# Autodesk Inventor assembly: main body assembly
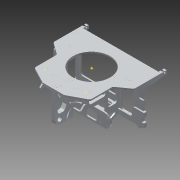
[picture p0: Inventor's stored thumbnail of the model, 180x180]
Saved by Autodesk Inventor 2015 (Build 190159000, 159)
## iProperties
Created: 2015-08-16
Part Number: main body assembly
Document SubType Name: Assembly
Designer: Thomas
Author: Thomas
## Documents named in this file (10)
- C:\Users\Thomas\Google Drive\MSc ROBOTICS\PROJECT\OpenROV\openrov-hardware\CAD_Files_OpenROV_v2_5\main body assembly.iam
- C:\Users\Thomas\Google Drive\MSc ROBOTICS\PROJECT\OpenROV\openrov-hardware\CAD_Files_OpenROV_v2_5\Internal Structure\Bulkhead 25083113.ipt
- C:\Users\Thomas\Google Drive\MSc ROBOTICS\PROJECT\OpenROV\openrov-hardware\CAD_Files_OpenROV_v2_5\Internal Structure\Axial Shroud Support 25090213.ipt
- C:\Users\Thomas\Google Drive\MSc ROBOTICS\PROJECT\OpenROV\openrov-hardware\CAD_Files_OpenROV_v2_5\Internal Structure\Bulkhead Brace 25100613.ipt
- C:\Users\Thomas\Google Drive\MSc ROBOTICS\PROJECT\OpenROV\openrov-hardware\CAD_Files_OpenROV_v2_5\Internal Structure\Vertical Motor Mount 25090213.ipt
- C:\Users\Thomas\Google Drive\MSc ROBOTICS\PROJECT\OpenROV\openrov-hardware\CAD_Files_OpenROV_v2_5\Internal Structure\Horizontal Motor Mount 25090213.ipt
- C:\Users\Thomas\Google Drive\MSc ROBOTICS\PROJECT\OpenROV\openrov-hardware\CAD_Files_OpenROV_v2_5\Internal Structure\Handle 25090213.ipt
- C:\Users\Thomas\Google Drive\MSc ROBOTICS\PROJECT\OpenROV\openrov-hardware\CAD_Files_OpenROV_v2_5\Internal Structure\Lateral Shroud Support 25090213.ipt
- C:\Users\Thomas\Google Drive\MSc ROBOTICS\PROJECT\OpenROV\openrov-hardware\CAD_Files_OpenROV_v2_5\Internal Structure\Top Plate 25090213.ipt
- C:\Users\Thomas\Google Drive\MSc ROBOTICS\PROJECT\OpenROV\openrov-hardware\CAD_Files_OpenROV_v2_5\Internal Structure\Tube Cradle 25090213.ipt
## Components (15 placed, 9 different names)
1. Bulkhead 25083113:1
2. Axial Shroud Support 25090213:1
3. Axial Shroud Support 25090213:2
4. Bulkhead Brace 25100613:1
5. Vertical Motor Mount 25090213:1
6. Horizontal Motor Mount 25090213:1
7. Handle 25090213:1
8. Handle 25090213:2
9. Handle 25090213:3
10. Lateral Shroud Support 25090213:1
11. Top Plate 25090213:1
12. Tube Cradle 25090213:1
13. Tube Cradle 25090213:2
14. Tube Cradle 25090213:3
15. Tube Cradle 25090213:4
## Relationships (42: Mate 31, Flush 11)
- [Mate]: Bulkhead 25083113:1 ↔ Axial Shroud Support 25090213:1
- [Mate]: Bulkhead 25083113:1 ↔ Axial Shroud Support 25090213:1
- [Mate]: Bulkhead 25083113:1 ↔ Axial Shroud Support 25090213:1
- [Mate]: Bulkhead 25083113:1 ↔ Axial Shroud Support 25090213:2
- [Mate]: Bulkhead 25083113:1 ↔ Axial Shroud Support 25090213:2
- [Mate]: Bulkhead 25083113:1 ↔ Axial Shroud Support 25090213:2
- [Mate]: Bulkhead 25083113:1 ↔ Bulkhead Brace 25100613:1
- [Flush]: Bulkhead 25083113:1 ↔ Bulkhead Brace 25100613:1
- [Flush]: Bulkhead 25083113:1 ↔ Bulkhead Brace 25100613:1
- [Mate]: Bulkhead 25083113:1 ↔ Vertical Motor Mount 25090213:1
- [Mate]: Bulkhead 25083113:1 ↔ Vertical Motor Mount 25090213:1
- [Mate]: Bulkhead 25083113:1 ↔ Vertical Motor Mount 25090213:1
- [Mate]: Vertical Motor Mount 25090213:1 ↔ Horizontal Motor Mount 25090213:1
- [Mate]: Vertical Motor Mount 25090213:1 ↔ Horizontal Motor Mount 25090213:1
- [Mate]: Vertical Motor Mount 25090213:1 ↔ Horizontal Motor Mount 25090213:1
- [Mate]: Handle 25090213:1 ↔ Handle 25090213:2
- [Flush]: Handle 25090213:1 ↔ Handle 25090213:2
- [Flush]: Handle 25090213:1 ↔ Handle 25090213:2
- [Mate]: Handle 25090213:2 ↔ Handle 25090213:3
- [Flush]: Handle 25090213:2 ↔ Handle 25090213:3
- [Flush]: Handle 25090213:2 ↔ Handle 25090213:3
- [Mate]: Handle 25090213:2 ↔ Lateral Shroud Support 25090213:1
- [Mate]: Handle 25090213:1 ↔ Lateral Shroud Support 25090213:1
- [Mate]: Handle 25090213:2 ↔ Lateral Shroud Support 25090213:1
- [Mate]: Handle 25090213:2 ↔ Top Plate 25090213:1
- [Flush]: Handle 25090213:2 ↔ Top Plate 25090213:1
- [Mate]: Handle 25090213:3 ↔ Top Plate 25090213:1
- [Mate]: Bulkhead 25083113:1 ↔ Top Plate 25090213:1
- [Mate]: Bulkhead 25083113:1 ↔ Top Plate 25090213:1
- [Mate]: Bulkhead 25083113:1 ↔ Top Plate 25090213:1
- [Mate]: Tube Cradle 25090213:1 ↔ Tube Cradle 25090213:2
- [Flush]: Tube Cradle 25090213:1 ↔ Tube Cradle 25090213:2
- [Flush]: Tube Cradle 25090213:1 ↔ Tube Cradle 25090213:2
- [Mate]: Tube Cradle 25090213:3 ↔ Tube Cradle 25090213:4
- [Flush]: Tube Cradle 25090213:3 ↔ Tube Cradle 25090213:4
- [Flush]: Tube Cradle 25090213:3 ↔ Tube Cradle 25090213:4
- [Mate]: Top Plate 25090213:1 ↔ Tube Cradle 25090213:2
- [Mate]: Bulkhead 25083113:1 ↔ Tube Cradle 25090213:2
- [Mate]: Bulkhead 25083113:1 ↔ Tube Cradle 25090213:2
- [Mate]: Top Plate 25090213:1 ↔ Tube Cradle 25090213:3
- [Mate]: Bulkhead 25083113:1 ↔ Tube Cradle 25090213:3
- [Mate]: Bulkhead 25083113:1 ↔ Tube Cradle 25090213:3
## Named parameters: d6_d39 = 0 mm, d7_d40 = 0 mm, d8_d41 = 0 mm
